# Autodesk Inventor assembly: am-0940a 6 HiGrip wheel REV2
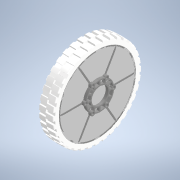
[picture p0: Inventor's stored thumbnail of the model, 180x180]
Saved by Autodesk Inventor 2020 (Build 240168000, 168)
## iProperties
Created: 2018-06-25
Part Number: am-0940a 6 HiGrip wheel REV2
Description: STEP AP214
Document SubType Name: Assembly
Designer: srini
Sending System: SolidWorks 2017
Preprocessor: SwSTEP 2.0
Title: am-0940a 6 HiGrip wheel REV2.STEP
Revision Number: ANY
## Documents named in this file (4)
- C:\Users\srini\Documents\FRC\2020\am-0940a 6 HiGrip wheel REV2.iam
- C:\Users\srini\Documents\FRC\2020\6 wheel Rev 4.ipt
- C:\Users\srini\Documents\FRC\2020\6 wheel tread II.ipt
- C:\Users\srini\Documents\FRC\2020\WheelMod6.ipt
## Components (3 placed, 3 different names)
1. 6 wheel Rev 4_1
2. 6 wheel tread II_2 — Flush:1
3. WheelMod6:1 — Flush:1
## Relationships (1: Flush 1)
- Flush:1: 6 wheel tread II_2 ↔ WheelMod6:1
